# Autodesk Inventor assembly: 万向节
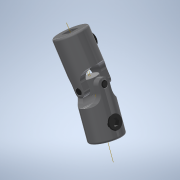
[picture p0: Inventor's stored thumbnail of the model, 180x180]
Saved by Autodesk Inventor 2020 (Build 240168000, 168)
## iProperties
Created: 2015-09-21
Part Number: 万向节
Material: 常规
Description: STEP AP214
Document SubType Name: Assembly
Designer: aresp
Sending System: SolidWorks 2015
Preprocessor: SwSTEP 2.0
Title: 276-2045-020 Rev2.STEP
Author: svradm
Revision Number: ANY
## Documents named in this file (3)
- C:\Users\aresp\Documents\Vault\常用部件库\vex原厂部件\万向节.iam
- C:\Users\aresp\Documents\Inventor\Content Center Files\R2020\zh-CN\万向节零件\常规.ipt
- C:\Users\aresp\Documents\Inventor\Content Center Files\R2020\zh-CN\万向节零件 中间连接\常规.ipt
## Components (3 placed, 2 different names)
1. 万向节零件 常规:1 — 配合:1, 相切:1, 配合:4
2. 万向节零件 常规:2 — 配合:2, 相切:2, 配合:3
3. 万向节零件 中间连接 常规:1 — 配合:1, 配合:2, 相切:1, 相切:2
## Relationships (6: Mate 4, Tangent 2)
- 配合:1 [Mate]: 万向节零件 常规:1 ↔ 万向节零件 中间连接 常规:1
- 配合:2 [Mate]: 万向节零件 常规:2 ↔ 万向节零件 中间连接 常规:1
- 相切:1 [Tangent] (0.127 mm): 万向节零件 常规:1 ↔ 万向节零件 中间连接 常规:1
- 相切:2 [Tangent] (0.127 mm): 万向节零件 常规:2 ↔ 万向节零件 中间连接 常规:1
- 配合:3 [Mate]: 万向节零件 常规:2
- 配合:4 [Mate]: 万向节零件 常规:1
